# Autodesk Inventor assembly: ploter
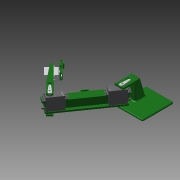
[picture p0: Inventor's stored thumbnail of the model, 180x180]
Saved by Autodesk Inventor 2013 (Build 170138000, 138)
## iProperties
Created: 2013-03-06
Part Number: ploter
Document SubType Name: Assembly
Designer: Masta
Author: Masta
## Documents named in this file (11)
- D:\rysownik\3D models\ploter.iam
- D:\rysownik\3D models\arm1.ipt
- D:\rysownik\3D models\serwo HK15138.ipt
- D:\rysownik\3D models\servo arm HK15138 2 cut to 1.ipt
- D:\rysownik\3D models\arm1a.ipt
- D:\rysownik\3D models\625ZZ.ipt
- D:\rysownik\3D models\base.ipt
- D:\rysownik\3D models\arm2.ipt
- D:\rysownik\3D models\hand1.ipt
- D:\rysownik\3D models\hand2.ipt
- D:\rysownik\3D models\serwo HK15148.ipt
## Components (14 placed, 10 different names)
1. arm1:1 — Insert:1, Insert:2, Insert:3, Insert:4
2. serwo HK15138:1 — Insert:2, Insert:3, Insert:5, Mate:1, Mate:2, Mate:3
3. serwo HK15138:2 — Insert:1, Insert:4, Insert:6
4. servo arm HK15138 2 cut to 1:1 — Insert:5, Insert:21
5. servo arm HK15138 2 cut to 1:2 — Insert:6, Insert:10
6. arm1a:1 — Mate:1, Mate:2, Insert:7, Insert:8, Mate:3
7. 625ZZ:1 — Insert:7, Insert:11
8. 625ZZ:2 — Insert:8, Insert:9
9. base:1 — Insert:9, Insert:10, Mate:4
10. arm2:1 — Insert:11, Insert:19, Insert:20, Insert:21
11. hand1:1 — Insert:15, Insert:16
12. hand2:1 — Insert:17, Insert:18
13. serwo HK15148:1 — Insert:14, Insert:19, Insert:20
14. servo arm HK15138 2 cut to 1:3 — Insert:14, Insert:15, Insert:16, Insert:17, Insert:18
## Relationships (23: Insert 19, Mate 4)
- Insert:1: arm1:1 ↔ serwo HK15138:2
- Insert:2: arm1:1 ↔ serwo HK15138:1
- Insert:3: arm1:1 ↔ serwo HK15138:1
- Insert:4: arm1:1 ↔ serwo HK15138:2
- Insert:5: serwo HK15138:1 ↔ servo arm HK15138 2 cut to 1:1
- Insert:6: serwo HK15138:2 ↔ servo arm HK15138 2 cut to 1:2
- Mate:1: serwo HK15138:1 ↔ arm1a:1
- Mate:2: serwo HK15138:1 ↔ arm1a:1
- Insert:7: arm1a:1 ↔ 625ZZ:1
- Insert:8: arm1a:1 ↔ 625ZZ:2
- Insert:9: 625ZZ:2 ↔ base:1
- Mate:3: serwo HK15138:1 ↔ arm1a:1
- Insert:10: servo arm HK15138 2 cut to 1:2 ↔ base:1
- Insert:11: 625ZZ:1 ↔ arm2:1
- Insert:14: serwo HK15148:1 ↔ servo arm HK15138 2 cut to 1:3
- Insert:15: hand1:1 ↔ servo arm HK15138 2 cut to 1:3
- Insert:16: hand1:1 ↔ servo arm HK15138 2 cut to 1:3
- Insert:17: hand2:1 ↔ servo arm HK15138 2 cut to 1:3
- Insert:18: hand2:1 ↔ servo arm HK15138 2 cut to 1:3
- Insert:19: arm2:1 ↔ serwo HK15148:1
- Insert:20: arm2:1 ↔ serwo HK15148:1
- Insert:21: servo arm HK15138 2 cut to 1:1 ↔ arm2:1
- Mate:4: base:1
